# Autodesk Inventor assembly: rapoukAssemblyv2
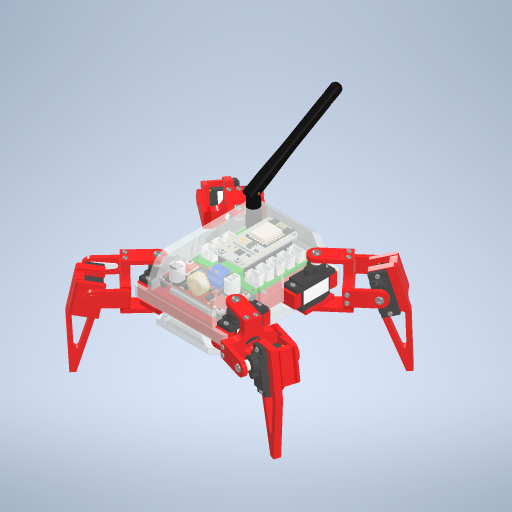
[picture p0: Inventor's stored thumbnail of the model, 512x512]
Saved by Autodesk Inventor 2024 (Build 280153000, 153)
## iProperties
Created: 2024-02-06
Part Number: rapoukAssemblyv2
Document SubType Name: Weldment
Designer: Roman Suk
Weld Material: Welded Aluminum-6061
Author: Roman Suk
## Documents named in this file (20)
- C:\Users\Roman Suk\Documents\Ročníkovka SŠ\Technical documentation\Final\rapoukAssemblyv2.iam
- C:\Users\Roman Suk\Documents\Ročníkovka SŠ\Technical documentation\Final\rapoukBaseAssemblyv1.iam
- C:\Users\Roman Suk\Documents\Ročníkovka SŠ\Technical documentation\Final\сервопривод EMAX ES08MA.ipt
- C:\Users\Roman Suk\Documents\Ročníkovka SŠ\Technical documentation\Final\rapoukMotherboardSuppportv0.ipt
- C:\Users\Roman Suk\Documents\Ročníkovka SŠ\Technical documentation\Final\XL4015 StepDown DC-DC 5A (CC-CV) v1\XL4015 StepDown DC-DC 5A (CC-CV) v1.iam
- C:\Users\Roman Suk\Documents\Ročníkovka SŠ\Technical documentation\Final\rapoukMotherboardAssemblyv0.iam
- C:\Users\Roman Suk\Documents\Ročníkovka SŠ\Technical documentation\Final\1assemble antenn\1assemble antenn.iam
- C:\Users\Roman Suk\Documents\Ročníkovka SŠ\Technical documentation\Final\ESP8266 v7\ESP8266 v7.iam
- C:\Users\Roman Suk\Documents\Ročníkovka SŠ\Technical documentation\Final\rapoukMiddleLegAssemblyv0.iam
- C:\Users\Roman Suk\Documents\Ročníkovka SŠ\Technical documentation\Final\rapoukLegAssemblyv0.iam
- C:\Users\Roman Suk\Documents\Ročníkovka SŠ\Technical documentation\Final\rapoukServoLegv0.ipt
- C:\Users\Roman Suk\Documents\Ročníkovka SŠ\Technical documentation\Final\rapoukMiddleLeg2v3.ipt
- C:\Users\Roman Suk\Documents\Ročníkovka SŠ\Technical documentation\Final\Bateria 18650.ipt
- C:\Users\Roman Suk\Documents\Ročníkovka SŠ\Technical documentation\Final\rapoukUSBChargerv0.ipt
- C:\Users\Roman Suk\Documents\Ročníkovka SŠ\Technical documentation\Final\rapoukBottomAssemblyv0.iam
- C:\Users\Roman Suk\Documents\Ročníkovka SŠ\Technical documentation\Final\M2 Nut v2.ipt
- C:\Users\Roman Suk\Documents\Ročníkovka SŠ\Technical documentation\Final\rapoukHexagonScrewM2×20v0.ipt
- C:\Users\Roman Suk\Documents\Ročníkovka SŠ\Technical documentation\Final\rapoukHexagonScrewM2,5v0.ipt
- C:\Users\Roman Suk\Documents\Ročníkovka SŠ\Technical documentation\Final\rapoukHexagonScrewM2v0.ipt
- C:\Users\Roman Suk\Documents\Ročníkovka SŠ\Technical documentation\Final\rapoukTopCoverv2.ipt
## Components (94 placed, 19 different names)
1. rapoukBaseAssemblyv1:1 [sub-assembly] — Insert:1, Insert:2, Insert:5, Insert:6, Insert:7, Insert:8, Insert:14, Insert:15, Tangent:20, Mate:40, Mate:44, Mate:45, Flush:5, Flush:6, Mate:46, Rotational:2, Rotational:4, Rotational:6, Rotational:8, Mate:66, Insert:37, Insert:38, Mate:67, Insert:39, Insert:40, Mate:69, Insert:41, Insert:42, Mate:70, Insert:43, Insert:44, Insert:45, Insert:46, Flush:7, Mate:76, Mate:77
2. сервопривод EMAX ES08MA:1 — Mate:69, Insert:41, Insert:42, Rotational:13, Insert:83, Insert:86
3. сервопривод EMAX ES08MA:2 — Mate:70, Insert:43, Insert:44, Rotational:14, Insert:81, Insert:82
4. сервопривод EMAX ES08MA:3 — Mate:67, Insert:39, Insert:40, Rotational:16, Insert:63, Insert:64
5. сервопривод EMAX ES08MA:4 — Mate:66, Insert:37, Insert:38, Rotational:15, Insert:84, Insert:85
6. rapoukMotherboardSuppportv0:1 — Insert:8, Insert:9
7. rapoukMotherboardSuppportv0:2 — Insert:15, Insert:16
8. rapoukMotherboardSuppportv0:3 — Insert:2, Insert:18
9. rapoukMotherboardSuppportv0:4 — Insert:14, Insert:17
10. rapoukMotherboardSuppportv0:5 — Insert:5, Insert:10
11. rapoukMotherboardSuppportv0:6 — Insert:6, Insert:11
12. rapoukMotherboardSuppportv0:7 — Insert:7, Insert:12
13. rapoukMotherboardSuppportv0:8 — Insert:1, Insert:13
14. XL4015 StepDown DC-DC 5A (CC-CV) v1:1 [sub-assembly] — Insert:9, Insert:10, Insert:11, Insert:12, Mate:43
15. rapoukMotherboardAssemblyv0:1 [sub-assembly] — Insert:13, Insert:16, Insert:17, Insert:18, Mate:14, Flush:1, Mate:15, Mate:16, Mate:17, Mate:18, Tangent:17, Tangent:18
16. 1assemble antenn:1 [sub-assembly] — Mate:14, Flush:1, Mate:15
17. ESP8266 v7:1 [sub-assembly] — Mate:16, Mate:17, Mate:18
18. rapoukMiddleLegAssemblyv0:3 [sub-assembly] — Insert:21, Insert:22, Insert:23, Insert:24, Rotational:1, Rotational:2
19. rapoukLegAssemblyv0:4 [sub-assembly] — Mate:21, Mate:26, Mate:30, Rotational:1
20. сервопривод EMAX ES08MA:7 — Mate:21, Mate:26, Mate:30, Rotational:9, Insert:71, Insert:72
21. rapoukServoLegv0:4 — Mate:33, Tangent:15, Tangent:16
22. rapoukMiddleLeg2v3:3 — Mate:33, Tangent:15, Tangent:16, Insert:23, Insert:24, Rotational:14, Insert:49, Insert:75, Insert:76
23. rapoukMiddleLeg2v3:5 — Insert:21, Insert:22, Rotational:9, Tangent:29, Tangent:30, Mate:64, Insert:52, Insert:73, Insert:74
24. Bateria 18650:1 — Tangent:17, Tangent:19, Flush:4, Mate:40
25. Bateria 18650:2 — Tangent:18, Tangent:19, Flush:4, Tangent:20
26. rapoukUSBChargerv0:1 — Mate:43, Mate:44, Mate:45
27. rapoukBottomAssemblyv0:1 [sub-assembly] — Flush:5, Flush:6, Mate:46, Mate:47, Mate:48, Mate:49, Mate:50
28. M2 Nut v2:1 — Mate:49, Mate:50, Mate:74
29. M2 Nut v2:2 — Mate:47, Mate:48, Mate:75
30. rapoukMiddleLegAssemblyv0:4 [sub-assembly] — Rotational:4
31. rapoukLegAssemblyv0:5 [sub-assembly]
32. сервопривод EMAX ES08MA:8 — Rotational:10, Insert:69, Insert:70
33. rapoukMiddleLeg2v3:6 — Rotational:13, Mate:73, Tangent:37, Tangent:38, Insert:50, Insert:67, Insert:68
34. rapoukMiddleLeg2v3:7 — Rotational:10, Insert:51, Insert:65, Insert:66
35. rapoukServoLegv0:9
36. rapoukMiddleLegAssemblyv0:5 [sub-assembly] — Rotational:6
37. rapoukLegAssemblyv0:6 [sub-assembly]
38. сервопривод EMAX ES08MA:9 — Rotational:12, Insert:77, Insert:78
39. rapoukMiddleLeg2v3:8 — Rotational:16, Mate:71, Tangent:35, Tangent:36, Insert:48, Insert:59, Insert:60
40. rapoukMiddleLeg2v3:9 — Rotational:12, Tangent:31, Tangent:32, Mate:65, Insert:53, Insert:61, Insert:62
41. rapoukMiddleLegAssemblyv0:6 [sub-assembly] — Rotational:8
42. rapoukLegAssemblyv0:7 [sub-assembly]
43. сервопривод EMAX ES08MA:10 — Rotational:11, Insert:79, Insert:80
44. rapoukMiddleLeg2v3:10 — Rotational:15, Mate:72, Tangent:33, Tangent:34, Insert:47, Insert:55, Insert:56
45. rapoukMiddleLeg2v3:11 — Rotational:11, Insert:54, Insert:57, Insert:58
46. rapoukServoLegv0:11
47. rapoukServoLegv0:12 — Tangent:29, Tangent:30, Mate:64
48. rapoukServoLegv0:13 — Tangent:31, Tangent:32, Mate:65
49. rapoukServoLegv0:14 — Mate:71, Tangent:35, Tangent:36
50. rapoukServoLegv0:15 — Mate:72, Tangent:33, Tangent:34
51. rapoukServoLegv0:17 — Mate:73, Tangent:37, Tangent:38
52. rapoukHexagonScrewM2×20v0:1 — Insert:46, Mate:74
53. rapoukHexagonScrewM2×20v0:2 — Insert:45, Mate:75
54. rapoukHexagonScrewM2,5v0:1 — Insert:50
55. rapoukHexagonScrewM2,5v0:2 — Insert:49
56. rapoukHexagonScrewM2,5v0:3 — Insert:48
57. rapoukHexagonScrewM2,5v0:4 — Insert:47
58. rapoukHexagonScrewM2,5v0:5 — Insert:54
59. rapoukHexagonScrewM2,5v0:6 — Insert:53
60. rapoukHexagonScrewM2,5v0:7 — Insert:52
61. rapoukHexagonScrewM2,5v0:8 — Insert:51
62. rapoukHexagonScrewM2v0:1 — Insert:58
63. rapoukHexagonScrewM2v0:2 — Insert:57
64. rapoukHexagonScrewM2v0:3 — Insert:56
65. rapoukHexagonScrewM2v0:4 — Insert:55
66. rapoukHexagonScrewM2v0:5 — Insert:62
67. rapoukHexagonScrewM2v0:6 — Insert:61
68. rapoukHexagonScrewM2v0:7 — Insert:60
69. rapoukHexagonScrewM2v0:8 — Insert:59
70. rapoukHexagonScrewM2v0:9 — Insert:64
71. rapoukHexagonScrewM2v0:10 — Insert:63
72. rapoukHexagonScrewM2v0:11 — Insert:69
73. rapoukHexagonScrewM2v0:12 — Insert:65
74. rapoukHexagonScrewM2v0:13 — Insert:66
75. rapoukHexagonScrewM2v0:14 — Insert:67
76. rapoukHexagonScrewM2v0:15 — Insert:70
77. rapoukHexagonScrewM2v0:16 — Insert:68
78. rapoukHexagonScrewM2v0:17 — Insert:71
79. rapoukHexagonScrewM2v0:18 — Insert:72
80. rapoukHexagonScrewM2v0:19 — Insert:74
81. rapoukHexagonScrewM2v0:20 — Insert:75
82. rapoukHexagonScrewM2v0:21 — Insert:76
83. rapoukHexagonScrewM2v0:22 — Insert:73
84. rapoukHexagonScrewM2v0:23 — Insert:77
85. rapoukHexagonScrewM2v0:24 — Insert:78
86. rapoukHexagonScrewM2v0:25 — Insert:80
87. rapoukHexagonScrewM2v0:26 — Insert:79
88. rapoukHexagonScrewM2v0:27 — Insert:84
89. rapoukHexagonScrewM2v0:28 — Insert:83
90. rapoukHexagonScrewM2v0:29 — Insert:85
91. rapoukHexagonScrewM2v0:30 — Insert:86
92. rapoukHexagonScrewM2v0:31 — Insert:82
93. rapoukHexagonScrewM2v0:32 — Insert:81
94. rapoukTopCoverv2:1 — Flush:7, Mate:76, Mate:77
## Relationships (165: Insert 82, Mate 42, Tangent 20, RevoluteJoint 16, Flush 5)
- Insert:1: rapoukBaseAssemblyv1:1 ↔ rapoukMotherboardSuppportv0:8
- Insert:2: rapoukBaseAssemblyv1:1 ↔ rapoukMotherboardSuppportv0:3
- Insert:5: rapoukBaseAssemblyv1:1 ↔ rapoukMotherboardSuppportv0:5
- Insert:6: rapoukBaseAssemblyv1:1 ↔ rapoukMotherboardSuppportv0:6
- Insert:7: rapoukBaseAssemblyv1:1 ↔ rapoukMotherboardSuppportv0:7
- Insert:8: rapoukBaseAssemblyv1:1 ↔ rapoukMotherboardSuppportv0:1
- Insert:9: rapoukMotherboardSuppportv0:1 ↔ XL4015 StepDown DC-DC 5A (CC-CV) v1:1
- Insert:10: rapoukMotherboardSuppportv0:5 ↔ XL4015 StepDown DC-DC 5A (CC-CV) v1:1
- Insert:11: rapoukMotherboardSuppportv0:6 ↔ XL4015 StepDown DC-DC 5A (CC-CV) v1:1
- Insert:12: rapoukMotherboardSuppportv0:7 ↔ XL4015 StepDown DC-DC 5A (CC-CV) v1:1
- Insert:13: rapoukMotherboardSuppportv0:8 ↔ rapoukMotherboardAssemblyv0:1
- Insert:14: rapoukBaseAssemblyv1:1 ↔ rapoukMotherboardSuppportv0:4
- Insert:15: rapoukBaseAssemblyv1:1 ↔ rapoukMotherboardSuppportv0:2
- Insert:16: rapoukMotherboardSuppportv0:2 ↔ rapoukMotherboardAssemblyv0:1
- Insert:17: rapoukMotherboardSuppportv0:4 ↔ rapoukMotherboardAssemblyv0:1
- Insert:18: rapoukMotherboardSuppportv0:3 ↔ rapoukMotherboardAssemblyv0:1
- Mate:14: rapoukMotherboardAssemblyv0:1 ↔ 1assemble antenn:1
- Flush:1 (-5 mm): rapoukMotherboardAssemblyv0:1 ↔ 1assemble antenn:1
- Mate:15 (-4 mm): rapoukMotherboardAssemblyv0:1 ↔ 1assemble antenn:1
- Mate:16: rapoukMotherboardAssemblyv0:1 ↔ ESP8266 v7:1
- Mate:17: rapoukMotherboardAssemblyv0:1 ↔ ESP8266 v7:1
- Mate:18: rapoukMotherboardAssemblyv0:1 ↔ ESP8266 v7:1
- Mate:21: rapoukLegAssemblyv0:4 ↔ сервопривод EMAX ES08MA:7
- Mate:26: rapoukLegAssemblyv0:4 ↔ сервопривод EMAX ES08MA:7
- Mate:30: rapoukLegAssemblyv0:4 ↔ сервопривод EMAX ES08MA:7
- Mate:33: rapoukServoLegv0:4 ↔ rapoukMiddleLeg2v3:3
- Tangent:15: rapoukServoLegv0:4 ↔ rapoukMiddleLeg2v3:3
- Tangent:16: rapoukServoLegv0:4 ↔ rapoukMiddleLeg2v3:3
- Tangent:17: rapoukMotherboardAssemblyv0:1 ↔ Bateria 18650:1
- Tangent:18: rapoukMotherboardAssemblyv0:1 ↔ Bateria 18650:2
- Tangent:19: Bateria 18650:1 ↔ Bateria 18650:2
- Flush:4: Bateria 18650:1 ↔ Bateria 18650:2
- Tangent:20 (3 mm): rapoukBaseAssemblyv1:1 ↔ Bateria 18650:2
- Mate:40 (2 mm): rapoukBaseAssemblyv1:1 ↔ Bateria 18650:1
- Mate:43 (2 mm): XL4015 StepDown DC-DC 5A (CC-CV) v1:1 ↔ rapoukUSBChargerv0:1
- Mate:44 (5 mm): rapoukBaseAssemblyv1:1 ↔ rapoukUSBChargerv0:1
- Mate:45: rapoukBaseAssemblyv1:1 ↔ rapoukUSBChargerv0:1
- Flush:5: rapoukBaseAssemblyv1:1 ↔ rapoukBottomAssemblyv0:1
- Flush:6: rapoukBaseAssemblyv1:1 ↔ rapoukBottomAssemblyv0:1
- Mate:46: rapoukBaseAssemblyv1:1 ↔ rapoukBottomAssemblyv0:1
- Mate:47: rapoukBottomAssemblyv0:1 ↔ M2 Nut v2:2
- Mate:48: rapoukBottomAssemblyv0:1 ↔ M2 Nut v2:2
- Mate:49: rapoukBottomAssemblyv0:1 ↔ M2 Nut v2:1
- Mate:50: rapoukBottomAssemblyv0:1 ↔ M2 Nut v2:1
- Insert:21: rapoukMiddleLegAssemblyv0:3 ↔ rapoukMiddleLeg2v3:5
- Insert:22: rapoukMiddleLegAssemblyv0:3 ↔ rapoukMiddleLeg2v3:5
- Insert:23: rapoukMiddleLegAssemblyv0:3 ↔ rapoukMiddleLeg2v3:3
- Insert:24: rapoukMiddleLegAssemblyv0:3 ↔ rapoukMiddleLeg2v3:3
- Rotational:1 [RevoluteJoint]: rapoukMiddleLegAssemblyv0:3 ↔ rapoukLegAssemblyv0:4
- Rotational:2 [RevoluteJoint] (0.5 mm): rapoukBaseAssemblyv1:1 ↔ rapoukMiddleLegAssemblyv0:3
- [Mate]: rapoukLegAssemblyv0:5 ↔ сервопривод EMAX ES08MA:8
- [Mate]: rapoukLegAssemblyv0:5 ↔ сервопривод EMAX ES08MA:8
- [Mate]: rapoukLegAssemblyv0:5 ↔ сервопривод EMAX ES08MA:8
- [Insert]: rapoukMiddleLegAssemblyv0:4 ↔ rapoukMiddleLeg2v3:7
- [Insert]: rapoukMiddleLegAssemblyv0:4 ↔ rapoukMiddleLeg2v3:7
- [Mate]: rapoukMiddleLeg2v3:7 ↔ rapoukServoLegv0:9
- [Tangent]: rapoukMiddleLeg2v3:7 ↔ rapoukServoLegv0:9
- [Tangent]: rapoukMiddleLeg2v3:7 ↔ rapoukServoLegv0:9
- [Insert]: rapoukMiddleLegAssemblyv0:4 ↔ rapoukMiddleLeg2v3:6
- [Insert]: rapoukMiddleLegAssemblyv0:4 ↔ rapoukMiddleLeg2v3:6
- [RevoluteJoint]: rapoukMiddleLegAssemblyv0:4 ↔ rapoukLegAssemblyv0:5
- Rotational:4 [RevoluteJoint] (-0.5 mm): rapoukBaseAssemblyv1:1 ↔ rapoukMiddleLegAssemblyv0:4
- [Mate]: rapoukLegAssemblyv0:6 ↔ сервопривод EMAX ES08MA:9
- [Mate]: rapoukLegAssemblyv0:6 ↔ сервопривод EMAX ES08MA:9
- [Mate]: rapoukLegAssemblyv0:6 ↔ сервопривод EMAX ES08MA:9
- [Insert]: rapoukMiddleLegAssemblyv0:5 ↔ rapoukMiddleLeg2v3:9
- [Insert]: rapoukMiddleLegAssemblyv0:5 ↔ rapoukMiddleLeg2v3:9
- [Insert]: rapoukMiddleLegAssemblyv0:5 ↔ rapoukMiddleLeg2v3:8
- [Insert]: rapoukMiddleLegAssemblyv0:5 ↔ rapoukMiddleLeg2v3:8
- [RevoluteJoint]: rapoukMiddleLegAssemblyv0:5 ↔ rapoukLegAssemblyv0:6
- Rotational:6 [RevoluteJoint] (-0.5 mm): rapoukBaseAssemblyv1:1 ↔ rapoukMiddleLegAssemblyv0:5
- [Mate]: rapoukLegAssemblyv0:7 ↔ сервопривод EMAX ES08MA:10
- [Mate]: rapoukLegAssemblyv0:7 ↔ сервопривод EMAX ES08MA:10
- [Mate]: rapoukLegAssemblyv0:7 ↔ сервопривод EMAX ES08MA:10
- [Insert]: rapoukMiddleLegAssemblyv0:6 ↔ rapoukMiddleLeg2v3:11
- [Insert]: rapoukMiddleLegAssemblyv0:6 ↔ rapoukMiddleLeg2v3:11
- [Mate]: rapoukMiddleLeg2v3:11 ↔ rapoukServoLegv0:11
- [Tangent]: rapoukMiddleLeg2v3:11 ↔ rapoukServoLegv0:11
- [Tangent]: rapoukMiddleLeg2v3:11 ↔ rapoukServoLegv0:11
- [Insert]: rapoukMiddleLegAssemblyv0:6 ↔ rapoukMiddleLeg2v3:10
- [Insert]: rapoukMiddleLegAssemblyv0:6 ↔ rapoukMiddleLeg2v3:10
- [RevoluteJoint]: rapoukMiddleLegAssemblyv0:6 ↔ rapoukLegAssemblyv0:7
- Rotational:8 [RevoluteJoint] (0.5 mm): rapoukBaseAssemblyv1:1 ↔ rapoukMiddleLegAssemblyv0:6
- Rotational:9 [RevoluteJoint] (-4.3 mm): сервопривод EMAX ES08MA:7 ↔ rapoukMiddleLeg2v3:5
- Tangent:29: rapoukMiddleLeg2v3:5 ↔ rapoukServoLegv0:12
- Tangent:30: rapoukMiddleLeg2v3:5 ↔ rapoukServoLegv0:12
- Mate:64: rapoukMiddleLeg2v3:5 ↔ rapoukServoLegv0:12
- Rotational:10 [RevoluteJoint] (4.3 mm): сервопривод EMAX ES08MA:8 ↔ rapoukMiddleLeg2v3:7
- Rotational:11 [RevoluteJoint] (-4.3 mm): сервопривод EMAX ES08MA:10 ↔ rapoukMiddleLeg2v3:11
- Rotational:12 [RevoluteJoint] (-4.3 mm): сервопривод EMAX ES08MA:9 ↔ rapoukMiddleLeg2v3:9
- Tangent:31: rapoukMiddleLeg2v3:9 ↔ rapoukServoLegv0:13
- Tangent:32: rapoukMiddleLeg2v3:9 ↔ rapoukServoLegv0:13
- Mate:65: rapoukMiddleLeg2v3:9 ↔ rapoukServoLegv0:13
- Mate:66: rapoukBaseAssemblyv1:1 ↔ сервопривод EMAX ES08MA:4
- Insert:37: rapoukBaseAssemblyv1:1 ↔ сервопривод EMAX ES08MA:4
- Insert:38: rapoukBaseAssemblyv1:1 ↔ сервопривод EMAX ES08MA:4
- Mate:67: rapoukBaseAssemblyv1:1 ↔ сервопривод EMAX ES08MA:3
- Insert:39: rapoukBaseAssemblyv1:1 ↔ сервопривод EMAX ES08MA:3
- Insert:40: rapoukBaseAssemblyv1:1 ↔ сервопривод EMAX ES08MA:3
- Mate:69: rapoukBaseAssemblyv1:1 ↔ сервопривод EMAX ES08MA:1
- Insert:41: rapoukBaseAssemblyv1:1 ↔ сервопривод EMAX ES08MA:1
- Insert:42: rapoukBaseAssemblyv1:1 ↔ сервопривод EMAX ES08MA:1
- Mate:70: rapoukBaseAssemblyv1:1 ↔ сервопривод EMAX ES08MA:2
- Insert:43: rapoukBaseAssemblyv1:1 ↔ сервопривод EMAX ES08MA:2
- Insert:44: rapoukBaseAssemblyv1:1 ↔ сервопривод EMAX ES08MA:2
- Rotational:13 [RevoluteJoint] (4.3 mm): сервопривод EMAX ES08MA:1 ↔ rapoukMiddleLeg2v3:6
- Rotational:14 [RevoluteJoint] (4.3 mm): сервопривод EMAX ES08MA:2 ↔ rapoukMiddleLeg2v3:3
- Rotational:15 [RevoluteJoint] (4.3 mm): сервопривод EMAX ES08MA:4 ↔ rapoukMiddleLeg2v3:10
- Rotational:16 [RevoluteJoint] (4.3 mm): сервопривод EMAX ES08MA:3 ↔ rapoukMiddleLeg2v3:8
- Mate:71: rapoukMiddleLeg2v3:8 ↔ rapoukServoLegv0:14
- Mate:72: rapoukMiddleLeg2v3:10 ↔ rapoukServoLegv0:15
- Tangent:33: rapoukMiddleLeg2v3:10 ↔ rapoukServoLegv0:15
- Tangent:34: rapoukMiddleLeg2v3:10 ↔ rapoukServoLegv0:15
- Tangent:35: rapoukMiddleLeg2v3:8 ↔ rapoukServoLegv0:14
- Tangent:36: rapoukMiddleLeg2v3:8 ↔ rapoukServoLegv0:14
- Mate:73: rapoukMiddleLeg2v3:6 ↔ rapoukServoLegv0:17
- Tangent:37: rapoukMiddleLeg2v3:6 ↔ rapoukServoLegv0:17
- Tangent:38: rapoukMiddleLeg2v3:6 ↔ rapoukServoLegv0:17
- Insert:45: rapoukBaseAssemblyv1:1 ↔ rapoukHexagonScrewM2×20v0:2
- Insert:46: rapoukBaseAssemblyv1:1 ↔ rapoukHexagonScrewM2×20v0:1
- Mate:74: M2 Nut v2:1 ↔ rapoukHexagonScrewM2×20v0:1
- Mate:75: M2 Nut v2:2 ↔ rapoukHexagonScrewM2×20v0:2
- Insert:47: rapoukMiddleLeg2v3:10 ↔ rapoukHexagonScrewM2,5v0:4
- Insert:48: rapoukMiddleLeg2v3:8 ↔ rapoukHexagonScrewM2,5v0:3
- Insert:49: rapoukMiddleLeg2v3:3 ↔ rapoukHexagonScrewM2,5v0:2
- Insert:50: rapoukMiddleLeg2v3:6 ↔ rapoukHexagonScrewM2,5v0:1
- Insert:51: rapoukMiddleLeg2v3:7 ↔ rapoukHexagonScrewM2,5v0:8
- Insert:52: rapoukMiddleLeg2v3:5 ↔ rapoukHexagonScrewM2,5v0:7
- Insert:53: rapoukMiddleLeg2v3:9 ↔ rapoukHexagonScrewM2,5v0:6
- Insert:54: rapoukMiddleLeg2v3:11 ↔ rapoukHexagonScrewM2,5v0:5
- Insert:55: rapoukMiddleLeg2v3:10 ↔ rapoukHexagonScrewM2v0:4
- Insert:56: rapoukMiddleLeg2v3:10 ↔ rapoukHexagonScrewM2v0:3
- Insert:57: rapoukMiddleLeg2v3:11 ↔ rapoukHexagonScrewM2v0:2
- Insert:58: rapoukMiddleLeg2v3:11 ↔ rapoukHexagonScrewM2v0:1
- Insert:59: rapoukMiddleLeg2v3:8 ↔ rapoukHexagonScrewM2v0:8
- Insert:60: rapoukMiddleLeg2v3:8 ↔ rapoukHexagonScrewM2v0:7
- Insert:61: rapoukMiddleLeg2v3:9 ↔ rapoukHexagonScrewM2v0:6
- Insert:62: rapoukMiddleLeg2v3:9 ↔ rapoukHexagonScrewM2v0:5
- Insert:63: сервопривод EMAX ES08MA:3 ↔ rapoukHexagonScrewM2v0:10
- Insert:64: сервопривод EMAX ES08MA:3 ↔ rapoukHexagonScrewM2v0:9
- Insert:65: rapoukMiddleLeg2v3:7 ↔ rapoukHexagonScrewM2v0:12
- Insert:66: rapoukMiddleLeg2v3:7 ↔ rapoukHexagonScrewM2v0:13
- Insert:67: rapoukMiddleLeg2v3:6 ↔ rapoukHexagonScrewM2v0:14
- Insert:68: rapoukMiddleLeg2v3:6 ↔ rapoukHexagonScrewM2v0:16
- Insert:69: сервопривод EMAX ES08MA:8 ↔ rapoukHexagonScrewM2v0:11
- Insert:70: сервопривод EMAX ES08MA:8 ↔ rapoukHexagonScrewM2v0:15
- Insert:71: сервопривод EMAX ES08MA:7 ↔ rapoukHexagonScrewM2v0:17
- Insert:72: сервопривод EMAX ES08MA:7 ↔ rapoukHexagonScrewM2v0:18
- Insert:73: rapoukMiddleLeg2v3:5 ↔ rapoukHexagonScrewM2v0:22
- Insert:74: rapoukMiddleLeg2v3:5 ↔ rapoukHexagonScrewM2v0:19
- Insert:75: rapoukMiddleLeg2v3:3 ↔ rapoukHexagonScrewM2v0:20
- Insert:76: rapoukMiddleLeg2v3:3 ↔ rapoukHexagonScrewM2v0:21
- Insert:77: сервопривод EMAX ES08MA:9 ↔ rapoukHexagonScrewM2v0:23
- Insert:78: сервопривод EMAX ES08MA:9 ↔ rapoukHexagonScrewM2v0:24
- Insert:79: сервопривод EMAX ES08MA:10 ↔ rapoukHexagonScrewM2v0:26
- Insert:80: сервопривод EMAX ES08MA:10 ↔ rapoukHexagonScrewM2v0:25
- Insert:81: сервопривод EMAX ES08MA:2 ↔ rapoukHexagonScrewM2v0:32
- Insert:82: сервопривод EMAX ES08MA:2 ↔ rapoukHexagonScrewM2v0:31
- Insert:83: сервопривод EMAX ES08MA:1 ↔ rapoukHexagonScrewM2v0:28
- Insert:84: сервопривод EMAX ES08MA:4 ↔ rapoukHexagonScrewM2v0:27
- Insert:85: сервопривод EMAX ES08MA:4 ↔ rapoukHexagonScrewM2v0:29
- Insert:86: сервопривод EMAX ES08MA:1 ↔ rapoukHexagonScrewM2v0:30
- Flush:7: rapoukBaseAssemblyv1:1 ↔ rapoukTopCoverv2:1
- Mate:76: rapoukBaseAssemblyv1:1 ↔ rapoukTopCoverv2:1
- Mate:77: rapoukBaseAssemblyv1:1 ↔ rapoukTopCoverv2:1
## Named parameters: d151_d135 = 0 mm, d152_d136 = 0 mm, d153_d139 = 0 mm, d154_d140 = 0 mm, d155_d147 = 0 mm, d156_d148 = 100.953704 deg, d157_d60 = 0 mm, d158_d64 = 0 mm, d159_d131 = 0 mm, d160_d132 = 0 mm, d161_d134 = 0 mm, d162_d55 = 0 mm, d167_d139 = 0 mm, d168_d140 = 0 mm, d169_d147 = 0 mm, d170_d148 = 105.713773 deg, d171_d60 = 0 mm, d172_d64 = 0 mm, d173_d131 = 0 mm, d174_d132 = 0 mm, d176_d55 = 0 mm, d179_d135 = 0 mm, d180_d136 = 0 mm, d181_d139 = 0 mm, d182_d140 = 0 mm, d183_d147 = 0 mm, d184_d148 = 100.743768 deg, d185_d60 = 0 mm, d186_d64 = 0 mm, d187_d131 = 0 mm, d188_d132 = 0 mm, d189_d134 = 0 mm, d190_d55 = 0 mm
